# Autodesk Inventor assembly: Assembly
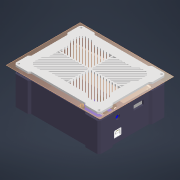
[picture p0: Inventor's stored thumbnail of the model, 180x180]
Saved by Autodesk Inventor 2021.1 (Build 251245010, 245A)
## iProperties
Created: 2020-11-26
Part Number: Assembly
Document SubType Name: Assembly
Designer: Alex
Author: Alex
## Documents named in this file (6)
- C:\Users\Alex\3D Objects\Inventor\Thermmolino2\Assembly.iam
- C:\Users\Alex\3D Objects\Inventor\Thermmolino2\Case.ipt
- C:\Users\Alex\3D Objects\Inventor\Thermmolino2\VFD_Mount.ipt
- C:\Users\Alex\3D Objects\Inventor\Thermmolino2\VFD_Dummy.ipt
- C:\Users\Alex\3D Objects\Inventor\Thermmolino2\Arduino\arduino uno.iam
- C:\Users\Alex\3D Objects\Inventor\Thermmolino2\Lid.ipt
## Components (5 placed, 5 different names)
1. Case:1 — Rotational:3, Rotational:4, Rotational:5, Flush:1
2. VFD_Mount:1 — Rotational:3, Rotational:4, Rotational:6, Rotational:7
3. arduino uno:1 [sub-assembly] — Rotational:5
4. VFD_Dummy:1 — Rotational:6, Rotational:7
5. Lid:1 — Flush:2
## Relationships (7: RevoluteJoint 5, Flush 2)
- Rotational:3 [RevoluteJoint]: Case:1 ↔ VFD_Mount:1
- Rotational:4 [RevoluteJoint]: Case:1 ↔ VFD_Mount:1
- Rotational:5 [RevoluteJoint]: Case:1 ↔ arduino uno:1
- Rotational:6 [RevoluteJoint]: VFD_Mount:1 ↔ VFD_Dummy:1
- Rotational:7 [RevoluteJoint]: VFD_Mount:1 ↔ VFD_Dummy:1
- Flush:1 (10 mm): Case:1
- Flush:2: Lid:1
